# Autodesk Inventor assembly: conish lagerblok test
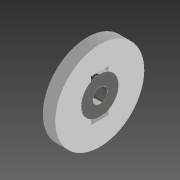
[picture p0: Inventor's stored thumbnail of the model, 180x180]
Saved by Autodesk Inventor 2020 (Build 240168000, 168)
## iProperties
Created: 2020-05-25
Part Number: conish lagerblok test
Document SubType Name: Assembly
Designer: stefa
Author: stefa
## Documents named in this file (3)
- D:\github_gedeeld\BeerMinder\3D-model\axis5_6\conish lagerblok test.iam
- D:\github_gedeeld\BeerMinder\3D-model\bearings\conische lager.ipt
- D:\github_gedeeld\BeerMinder\3D-model\axis5_6\conischLagerBlok.ipt
## Components (2 placed, 2 different names)
1. conische lager:1
2. conischLagerBlok:1 — Flush:1
## Relationships (1: Flush 1)
- Flush:1: conischLagerBlok:1
